# Autodesk Inventor assembly: Assembly_center_unit
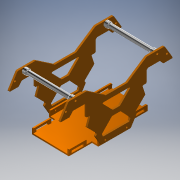
[picture p0: Inventor's stored thumbnail of the model, 180x180]
Saved by Autodesk Inventor 2018.1 (Build 221171000, 171)
## iProperties
Created: 2019-09-25
Part Number: Assembly_center_unit
Document SubType Name: Assembly
Designer: maste
Author: maste
## Documents named in this file (4)
- C:\Users\maste\Documents\GitHub\autobot\robot_model\Assembly_center_unit.iam
- C:\Users\maste\Documents\GitHub\autobot\robot_model\RCT-H112_stick_battery_plate.ipt
- C:\Users\maste\Documents\GitHub\autobot\robot_model\RCT-H001_Al_side_plate.ipt
- C:\Users\maste\Documents\GitHub\autobot\robot_model\RCT-H010_Al_side_plate_post.ipt
## Components (5 placed, 3 different names)
1. RCT-H112_stick_battery_plate:1 — Mate:1, Mate:2, Mate:3, Mate:4, Mate:5, Mate:6
2. RCT-H001_Al_side_plate:1 — Mate:1, Mate:2, Mate:3, Mate:7, Mate:8, Mate:9, Mate:10
3. RCT-H001_Al_side_plate:2 — Mate:4, Mate:5, Mate:6
4. RCT-H010_Al_side_plate_post:1 — Mate:7, Mate:8
5. RCT-H010_Al_side_plate_post:2 — Mate:9, Mate:10
## Relationships (10: Mate 10)
- Mate:1: RCT-H112_stick_battery_plate:1 ↔ RCT-H001_Al_side_plate:1
- Mate:2: RCT-H112_stick_battery_plate:1 ↔ RCT-H001_Al_side_plate:1
- Mate:3: RCT-H112_stick_battery_plate:1 ↔ RCT-H001_Al_side_plate:1
- Mate:4: RCT-H112_stick_battery_plate:1 ↔ RCT-H001_Al_side_plate:2
- Mate:5: RCT-H112_stick_battery_plate:1 ↔ RCT-H001_Al_side_plate:2
- Mate:6: RCT-H112_stick_battery_plate:1 ↔ RCT-H001_Al_side_plate:2
- Mate:7: RCT-H001_Al_side_plate:1 ↔ RCT-H010_Al_side_plate_post:1
- Mate:8: RCT-H001_Al_side_plate:1 ↔ RCT-H010_Al_side_plate_post:1
- Mate:9: RCT-H001_Al_side_plate:1 ↔ RCT-H010_Al_side_plate_post:2
- Mate:10: RCT-H001_Al_side_plate:1 ↔ RCT-H010_Al_side_plate_post:2
